# Autodesk Inventor assembly: MIRright脚四半
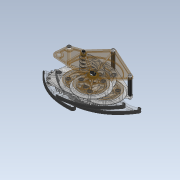
[picture p0: Inventor's stored thumbnail of the model, 180x180]
Saved by Autodesk Inventor 2020.2 (Build 242310000, 310)
## iProperties
Created: 2020-03-11
Part Number: MIRright脚四半
Document SubType Name: Assembly
Designer: aoyama
Mass: 222.66 g
Surface Area: 1659.29 cm^2
Volume: 108.119 cm^3
Density: 2.0594 g/cm^3
Author: aoyam
## Documents named in this file (38)
- C:\Users\aoyam\Desktop\SRDC_local\Inventor\二年機\Geminiβ\脚\MIR達\MIRright脚四半.iam
- C:\Users\aoyam\Desktop\SRDC_local\Inventor\二年機\Geminiβ\汎用部品\MIR達\MIRrightワッシャD8d6m0.5.ipt
- C:\Users\aoyam\Desktop\SRDC_local\Inventor\二年機\Geminiβ\汎用部品\MIR達\MIRrightスペーサーM3L30アルミ.ipt
- C:\Users\aoyam\Desktop\SRDC_local\Inventor\二年機\Geminiβ\汎用部品\MIR達\MIRrightネジボタンM3L6.ipt
- C:\Users\aoyam\Desktop\SRDC_local\Inventor\二年機\Geminiβ\汎用部品\MIR達\MIRrightネジボタンM3L8.ipt
- C:\Users\aoyam\Desktop\SRDC_local\Inventor\二年機\Geminiβ\汎用部品\MIR達\MIRrightスペーサーM3L30樹脂.ipt
- C:\Users\aoyam\Desktop\SRDC_local\Inventor\二年機\Geminiβ\汎用部品\MIR達\MIRrightネジアルミM3L6.ipt
- C:\Users\aoyam\Desktop\SRDC_local\Inventor\二年機\Geminiβ\脚\ネジクランク\MIR達\MIRright脚一枚.iam
- C:\Users\aoyam\Desktop\SRDC_local\Inventor\二年機\Geminiβ\脚\ネジクランク\MIR達\MIRrightカムL4F.ipt
- C:\Users\aoyam\Desktop\SRDC_local\Inventor\二年機\Geminiβ\汎用部品\MIR達\MIRrightオイレスドライメットFd10D12L3.ipt
- C:\Users\aoyam\Desktop\SRDC_local\Inventor\二年機\Geminiβ\汎用部品\MIR達\MIRrightｍ2歯数25ギアネジ.ipt
- C:\Users\aoyam\Desktop\SRDC_local\Inventor\二年機\Geminiβ\脚\ネジクランク\MIR達\MIRrightカムL3.ipt
- C:\Users\aoyam\Desktop\SRDC_local\Inventor\二年機\Geminiβ\汎用部品\MIR達\MIRrightオイレスドライメットFd10D12L4.ipt
- C:\Users\aoyam\Desktop\SRDC_local\Inventor\二年機\Geminiβ\脚\ネジクランク\MIR達\MIRrightカムL4.ipt
- C:\Users\aoyam\Desktop\SRDC_local\Inventor\二年機\Geminiβ\汎用部品\MIR達\MIRrightネジキャップM3L45.ipt
- C:\Users\aoyam\Desktop\SRDC_local\Inventor\二年機\Geminiβ\汎用部品\MIR達\MIRrightナットナイロンM3.ipt
- C:\Users\aoyam\Desktop\SRDC_local\Inventor\二年機\Geminiβ\汎用部品\MIR達\MIRrightスペーサーM3L40アルミ.ipt
- C:\Users\aoyam\Desktop\SRDC_local\Inventor\二年機\Geminiβ\汎用部品\MIR達\MIRrightネジキャップM3L15.ipt
- C:\Users\aoyam\Desktop\SRDC_local\Inventor\二年機\Geminiβ\脚\脚フレーム外側前.ipt
- C:\Users\aoyam\Desktop\SRDC_local\Inventor\二年機\Geminiβ\汎用部品\オイレスFd6D8L7.ipt
- C:\Users\aoyam\Desktop\SRDC_local\Inventor\二年機\Geminiβ\汎用部品\ネジ超極低頭M3L6.ipt
- C:\Users\aoyam\Desktop\SRDC_local\Inventor\二年機\Geminiβ\脚\脚フレーム内側前改弐.ipt
- C:\Users\aoyam\Desktop\SRDC_local\Inventor\二年機\Geminiβ\汎用部品\スペーサー中空M3L5樹脂.ipt
- C:\Users\aoyam\Desktop\SRDC_local\Inventor\二年機\Geminiβ\汎用部品\ネジ皿M3L8.ipt
- C:\Users\aoyam\Desktop\SRDC_local\Inventor\二年機\Geminiβ\汎用部品\スペーサー中空M3L4樹脂.ipt
- C:\Users\aoyam\Desktop\SRDC_local\Inventor\二年機\Geminiβ\汎用部品\ベアリングFd6D12B4.ipt
- C:\Users\aoyam\Desktop\SRDC_local\Inventor\二年機\Geminiβ\汎用部品\ベアリングFd4D11B4.ipt
- C:\Users\aoyam\Desktop\SRDC_local\Inventor\二年機\Geminiβ\汎用部品\ワッシャD7d4m0.5.ipt
- C:\Users\aoyam\Desktop\SRDC_local\Inventor\二年機\Geminiβ\汎用部品\ｍ2歯数17ギアd3.99.ipt
- C:\Users\aoyam\Desktop\SRDC_local\Inventor\二年機\Geminiβ\汎用部品\オイレスFd6D8L4.ipt
- C:\Users\aoyam\Desktop\SRDC_local\Inventor\二年機\Geminiβ\汎用部品\ワッシャD8d6m0.5.ipt
- C:\Users\aoyam\Desktop\SRDC_local\Inventor\二年機\Geminiβ\汎用部品\ｍ2歯数14ギアd12.ipt
- C:\Users\aoyam\Desktop\SRDC_local\Inventor\二年機\Geminiβ\汎用部品\ワッシャD10d6m0.3.ipt
- C:\Users\aoyam\Desktop\SRDC_local\Inventor\二年機\Geminiβ\汎用部品\オイレス外径8内径6L3.ipt
- C:\Users\aoyam\Desktop\SRDC_local\Inventor\二年機\Geminiβ\脚\MIRright脚ギアトレイン2.ipt
- C:\Users\aoyam\Desktop\SRDC_local\Inventor\二年機\Geminiβ\汎用部品\ネジボタンM3L10.ipt
- C:\Users\aoyam\Desktop\SRDC_local\Inventor\二年機\Geminiβ\汎用部品\平行ピンD4L12.ipt
- C:\Users\aoyam\Desktop\SRDC_local\Inventor\二年機\Geminiβ\汎用部品\ポリスラd6D14t0.25.ipt
## Components (62 placed, 37 different names)
1. MIRrightスペーサーM3L30アルミ:1 — 挿入:93, 挿入:84, 挿入:88, メイト:10, メイト:11, メイト:12, メイト:13, 挿入:100
2. MIRrightネジボタンM3L6:1 — 挿入:103
3. MIRrightネジボタンM3L8:1 — 挿入:85
4. MIRrightスペーサーM3L30樹脂:1 — 挿入:98, 挿入:108
5. MIRrightスペーサーM3L30樹脂:2 — 挿入:99
6. MIRrightワッシャD8d6m0.5:3 — 挿入:93, 挿入:129
7. MIRrightワッシャD8d6m0.5:4 — 挿入:130, 挿入:88
8. MIRrightワッシャD8d6m0.5:5 — 挿入:129
9. MIRrightネジアルミM3L6:1 — 挿入:102
10. MIRrightネジアルミM3L6:2 — 挿入:101
11. MIRrightネジアルミM3L6:3 — 挿入:86
12. MIRrightネジアルミM3L6:4 — 挿入:87
13. MIRright脚一枚:1 [sub-assembly] — 挿入:104, 挿入:103, 挿入:110, 挿入:109, メイト:13, 挿入:94
14. MIRright脚一枚:2 [sub-assembly] — 挿入:104, 挿入:103, 挿入:106, 挿入:105, メイト:12, 挿入:93
15. MIRright脚一枚:3 [sub-assembly] — 挿入:106, 挿入:105, 挿入:108, 挿入:107, メイト:11, 挿入:92
16. MIRright脚一枚:4 [sub-assembly] — 挿入:108, 挿入:107, メイト:6, メイト:7, メイト:10, 挿入:91
17. MIRrightカムL4F:1 — 挿入:110, 挿入:109, 挿入:112, 挿入:119, 挿入:120
18. MIRrightオイレスドライメットFd10D12L3:1 — 挿入:112, 挿入:89
19. MIRrightｍ2歯数25ギアネジ:1 — メイト:6, 挿入:114, 挿入:116, 挿入:115, メイト:15
20. MIRrightオイレスドライメットFd10D12L3:2 — 挿入:114
21. MIRrightカムL3:1 — 挿入:116, 挿入:115, 挿入:121, 挿入:122
22. MIRrightオイレスドライメットFd10D12L4:1 — 挿入:118, 挿入:107
23. MIRrightカムL4:1 — メイト:7, 挿入:118, メイト:15
24. MIRrightネジキャップM3L45:1 — 挿入:119, メイト:16
25. MIRrightネジキャップM3L45:2 — 挿入:120
26. MIRrightナットナイロンM3:1 — 挿入:121, メイト:8, メイト:16
27. MIRrightナットナイロンM3:2 — メイト:8, 挿入:122
28. MIRrightスペーサーM3L40アルミ:1 — 挿入:96, メイト:14, 挿入:114
29. MIRrightワッシャD8d6m0.5:6 — 挿入:130
30. MIRrightネジキャップM3L15:1 — 挿入:128
31. 脚フレーム外側前:1 — 挿入:84, 挿入:85, 挿入:86, 挿入:87, 挿入:89, メイト:14, 挿入:108
32. オイレスFd6D8L7:1 — 挿入:91
33. オイレスFd6D8L7:2 — 挿入:92
34. オイレスFd6D8L7:3 — 挿入:93
35. オイレスFd6D8L7:4 — 挿入:94
36. ネジ超極低頭M3L6:1 — 挿入:96
37. 脚フレーム内側前改弐:1 — 挿入:98, 挿入:99, 挿入:100, 挿入:101, 挿入:102, 挿入:103, 挿入:107, 挿入:109, 挿入:110, 挿入:111, 挿入:112, 挿入:113, 挿入:115, 挿入:120
38. スペーサー中空M3L5樹脂:1 — 挿入:109, 挿入:126
39. スペーサー中空M3L5樹脂:2 — 挿入:110, 挿入:127
40. スペーサー中空M3L5樹脂:3 — 挿入:111
41. スペーサー中空M3L5樹脂:4 — 挿入:112
42. ネジ皿M3L8:1 — 挿入:113
43. スペーサー中空M3L4樹脂:1 — 挿入:114
44. ベアリングFd6D12B4:1 — 挿入:122, 挿入:123, 挿入:124
45. ベアリングFd4D11B4:1 — 挿入:115, 挿入:116
46. ベアリングFd4D11B4:2 — 挿入:119, 挿入:133
47. ワッシャD7d4m0.5:1 — 挿入:118, 挿入:119
48. ワッシャD7d4m0.5:2 — 挿入:116, 挿入:117
49. ｍ2歯数17ギアd3.99:1 — 挿入:117, 挿入:118
50. オイレスFd6D8L4:1 — 挿入:120, 挿入:121
51. ワッシャD8d6m0.5:4 — 挿入:121, 挿入:123
52. ｍ2歯数14ギアd12:1 — 挿入:122
53. ワッシャD10d6m0.3:1 — 挿入:124
54. オイレス外径8内径6L3:1 — 挿入:135, 挿入:136
55. MIRright脚ギアトレイン2:1 — 挿入:126, 挿入:127, 挿入:128, 挿入:129, 挿入:130, 挿入:131, 挿入:132, 挿入:135
56. ネジボタンM3L10:1 — 挿入:129
57. ネジボタンM3L10:2 — 挿入:130
58. ネジボタンM3L10:3 — 挿入:131
59. ネジボタンM3L10:4 — 挿入:132
60. 平行ピンD4L12:1 — 挿入:133
61. ポリスラd6D14t0.25:1 — 挿入:134, 挿入:136
62. ポリスラd6D14t0.25:2 — 挿入:134
## Relationships (76: Insert 66, Mate 10)
- 挿入:93 [Insert]: MIRrightスペーサーM3L30アルミ:1 ↔ MIRrightワッシャD8d6m0.5:3
- 挿入:129 [Insert]: MIRrightワッシャD8d6m0.5:3 ↔ MIRrightワッシャD8d6m0.5:5
- 挿入:104 [Insert]: MIRright脚一枚:1 ↔ MIRright脚一枚:2
- 挿入:103 [Insert]: MIRright脚一枚:1 ↔ MIRright脚一枚:2
- 挿入:106 [Insert]: MIRright脚一枚:2 ↔ MIRright脚一枚:3
- 挿入:105 [Insert]: MIRright脚一枚:2 ↔ MIRright脚一枚:3
- 挿入:108 [Insert]: MIRright脚一枚:3 ↔ MIRright脚一枚:4
- 挿入:107 [Insert]: MIRright脚一枚:3 ↔ MIRright脚一枚:4
- 挿入:110 [Insert]: MIRright脚一枚:1 ↔ MIRrightカムL4F:1
- 挿入:109 [Insert]: MIRright脚一枚:1 ↔ MIRrightカムL4F:1
- 挿入:112 [Insert]: MIRrightカムL4F:1 ↔ MIRrightオイレスドライメットFd10D12L3:1
- メイト:6 [Mate]: MIRright脚一枚:4 ↔ MIRrightｍ2歯数25ギアネジ:1
- 挿入:114 [Insert]: MIRrightｍ2歯数25ギアネジ:1 ↔ MIRrightオイレスドライメットFd10D12L3:2
- 挿入:116 [Insert]: MIRrightｍ2歯数25ギアネジ:1 ↔ MIRrightカムL3:1
- 挿入:115 [Insert]: MIRrightｍ2歯数25ギアネジ:1 ↔ MIRrightカムL3:1
- メイト:7 [Mate]: MIRright脚一枚:4 ↔ MIRrightカムL4:1
- 挿入:118 [Insert]: MIRrightオイレスドライメットFd10D12L4:1 ↔ MIRrightカムL4:1
- 挿入:119 [Insert]: MIRrightカムL4F:1 ↔ MIRrightネジキャップM3L45:1
- 挿入:120 [Insert]: MIRrightカムL4F:1 ↔ MIRrightネジキャップM3L45:2
- 挿入:121 [Insert]: MIRrightカムL3:1 ↔ MIRrightナットナイロンM3:1
- メイト:8 [Mate]: MIRrightナットナイロンM3:1 ↔ MIRrightナットナイロンM3:2
- 挿入:122 [Insert]: MIRrightカムL3:1 ↔ MIRrightナットナイロンM3:2
- 挿入:130 [Insert]: MIRrightワッシャD8d6m0.5:4 ↔ MIRrightワッシャD8d6m0.5:6
- 挿入:84 [Insert]: MIRrightスペーサーM3L30アルミ:1 ↔ 脚フレーム外側前:1
- 挿入:85 [Insert]: MIRrightネジボタンM3L8:1 ↔ 脚フレーム外側前:1
- 挿入:86 [Insert]: MIRrightネジアルミM3L6:3 ↔ 脚フレーム外側前:1
- 挿入:87 [Insert]: MIRrightネジアルミM3L6:4 ↔ 脚フレーム外側前:1
- 挿入:88 [Insert]: MIRrightスペーサーM3L30アルミ:1 ↔ MIRrightワッシャD8d6m0.5:4
- 挿入:89 [Insert]: MIRrightオイレスドライメットFd10D12L3:1 ↔ 脚フレーム外側前:1
- メイト:10 [Mate]: MIRrightスペーサーM3L30アルミ:1 ↔ MIRright脚一枚:4
- メイト:11 [Mate]: MIRrightスペーサーM3L30アルミ:1 ↔ MIRright脚一枚:3
- メイト:12 [Mate]: MIRrightスペーサーM3L30アルミ:1 ↔ MIRright脚一枚:2
- メイト:13 [Mate]: MIRrightスペーサーM3L30アルミ:1 ↔ MIRright脚一枚:1
- 挿入:91 [Insert]: MIRright脚一枚:4 ↔ オイレスFd6D8L7:1
- 挿入:92 [Insert]: MIRright脚一枚:3 ↔ オイレスFd6D8L7:2
- 挿入:93 [Insert]: MIRright脚一枚:2 ↔ オイレスFd6D8L7:3
- 挿入:94 [Insert]: MIRright脚一枚:1 ↔ オイレスFd6D8L7:4
- 挿入:96 [Insert]: MIRrightスペーサーM3L40アルミ:1 ↔ ネジ超極低頭M3L6:1
- メイト:14 [Mate]: MIRrightスペーサーM3L40アルミ:1 ↔ 脚フレーム外側前:1
- 挿入:98 [Insert]: MIRrightスペーサーM3L30樹脂:1 ↔ 脚フレーム内側前改弐:1
- 挿入:99 [Insert]: MIRrightスペーサーM3L30樹脂:2 ↔ 脚フレーム内側前改弐:1
- 挿入:100 [Insert]: MIRrightスペーサーM3L30アルミ:1 ↔ 脚フレーム内側前改弐:1
- 挿入:101 [Insert]: MIRrightネジアルミM3L6:2 ↔ 脚フレーム内側前改弐:1
- 挿入:102 [Insert]: MIRrightネジアルミM3L6:1 ↔ 脚フレーム内側前改弐:1
- 挿入:103 [Insert]: MIRrightネジボタンM3L6:1 ↔ 脚フレーム内側前改弐:1
- 挿入:107 [Insert]: MIRrightオイレスドライメットFd10D12L4:1 ↔ 脚フレーム内側前改弐:1
- メイト:15 [Mate]: MIRrightｍ2歯数25ギアネジ:1 ↔ MIRrightカムL4:1
- メイト:16 [Mate]: MIRrightネジキャップM3L45:1 ↔ MIRrightナットナイロンM3:1
- 挿入:108 [Insert]: MIRrightスペーサーM3L30樹脂:1 ↔ 脚フレーム外側前:1
- 挿入:109 [Insert]: 脚フレーム内側前改弐:1 ↔ スペーサー中空M3L5樹脂:1
- 挿入:110 [Insert]: 脚フレーム内側前改弐:1 ↔ スペーサー中空M3L5樹脂:2
- 挿入:111 [Insert]: 脚フレーム内側前改弐:1 ↔ スペーサー中空M3L5樹脂:3
- 挿入:112 [Insert]: 脚フレーム内側前改弐:1 ↔ スペーサー中空M3L5樹脂:4
- 挿入:113 [Insert]: 脚フレーム内側前改弐:1 ↔ ネジ皿M3L8:1
- 挿入:114 [Insert]: MIRrightスペーサーM3L40アルミ:1 ↔ スペーサー中空M3L4樹脂:1
- 挿入:115 [Insert]: 脚フレーム内側前改弐:1 ↔ ベアリングFd4D11B4:1
- 挿入:116 [Insert]: ベアリングFd4D11B4:1 ↔ ワッシャD7d4m0.5:2
- 挿入:117 [Insert]: ワッシャD7d4m0.5:2 ↔ ｍ2歯数17ギアd3.99:1
- 挿入:118 [Insert]: ワッシャD7d4m0.5:1 ↔ ｍ2歯数17ギアd3.99:1
- 挿入:119 [Insert]: ベアリングFd4D11B4:2 ↔ ワッシャD7d4m0.5:1
- 挿入:120 [Insert]: 脚フレーム内側前改弐:1 ↔ オイレスFd6D8L4:1
- 挿入:121 [Insert]: オイレスFd6D8L4:1 ↔ ワッシャD8d6m0.5:4
- 挿入:122 [Insert]: ベアリングFd6D12B4:1 ↔ ｍ2歯数14ギアd12:1
- 挿入:123 [Insert]: ベアリングFd6D12B4:1 ↔ ワッシャD8d6m0.5:4
- 挿入:124 [Insert]: ベアリングFd6D12B4:1 ↔ ワッシャD10d6m0.3:1
- 挿入:126 [Insert]: スペーサー中空M3L5樹脂:1 ↔ MIRright脚ギアトレイン2:1
- 挿入:127 [Insert]: スペーサー中空M3L5樹脂:2 ↔ MIRright脚ギアトレイン2:1
- 挿入:128 [Insert]: MIRrightネジキャップM3L15:1 ↔ MIRright脚ギアトレイン2:1
- 挿入:129 [Insert]: MIRright脚ギアトレイン2:1 ↔ ネジボタンM3L10:1
- 挿入:130 [Insert]: MIRright脚ギアトレイン2:1 ↔ ネジボタンM3L10:2
- 挿入:131 [Insert]: MIRright脚ギアトレイン2:1 ↔ ネジボタンM3L10:3
- 挿入:132 [Insert]: MIRright脚ギアトレイン2:1 ↔ ネジボタンM3L10:4
- 挿入:133 [Insert]: ベアリングFd4D11B4:2 ↔ 平行ピンD4L12:1
- 挿入:134 [Insert]: ポリスラd6D14t0.25:1 ↔ ポリスラd6D14t0.25:2
- 挿入:135 [Insert]: オイレス外径8内径6L3:1 ↔ MIRright脚ギアトレイン2:1
- 挿入:136 [Insert]: オイレス外径8内径6L3:1 ↔ ポリスラd6D14t0.25:1
